# Autodesk Inventor assembly: 2020-2040_right
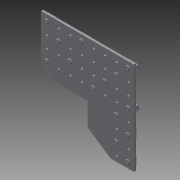
[picture p0: Inventor's stored thumbnail of the model, 180x180]
Saved by Autodesk Inventor 2014 (Build 180170000, 170)
## iProperties
Created: 2014-10-05
Part Number: 2020-2040_right
Document SubType Name: Assembly
Designer: Matthew
Author: Matthew
## Documents named in this file (3)
- C:\Users\Matthew\Documents\GitHub\CNC Mill\8020\2020-2040_right.iam
- C:\Users\Matthew\Documents\GitHub\CNC Mill\8020\2020-2040_mounting_plate.ipt
- C:\Users\Matthew\Documents\GitHub\CNC Mill\8020\0.5in_tnut.iam
## Components (15 placed, 2 different names)
1. 2020-2040_mounting_plate:1 — Insert:1, Insert:16, Insert:17, Insert:18, Insert:19, Insert:20, Insert:21, Insert:22, Insert:23, Insert:24, Insert:25, Insert:26, Insert:27, Insert:28
2. 0.5in_tnut:8 [sub-assembly] — Insert:17, Flush:2
3. 0.5in_tnut:13 [sub-assembly] — Insert:1
4. 0.5in_tnut:16 [sub-assembly] — Insert:16
5. 0.5in_tnut:18 [sub-assembly] — Insert:20, Flush:3
6. 0.5in_tnut:19 [sub-assembly] — Insert:18, Flush:3
7. 0.5in_tnut:20 [sub-assembly] — Insert:19, Flush:2
8. 0.5in_tnut:21 [sub-assembly] — Insert:21
9. 0.5in_tnut:22 [sub-assembly] — Insert:23
10. 0.5in_tnut:23 [sub-assembly] — Insert:22
11. 0.5in_tnut:24 [sub-assembly] — Insert:27
12. 0.5in_tnut:25 [sub-assembly] — Insert:26
13. 0.5in_tnut:26 [sub-assembly] — Insert:25
14. 0.5in_tnut:27 [sub-assembly] — Insert:24
15. 0.5in_tnut:28 [sub-assembly] — Insert:28
## Relationships (16: Insert 14, Flush 2)
- Insert:1: 2020-2040_mounting_plate:1 ↔ 0.5in_tnut:13
- Insert:16: 2020-2040_mounting_plate:1 ↔ 0.5in_tnut:16
- Insert:17: 2020-2040_mounting_plate:1 ↔ 0.5in_tnut:8
- Insert:18: 2020-2040_mounting_plate:1 ↔ 0.5in_tnut:19
- Insert:19: 2020-2040_mounting_plate:1 ↔ 0.5in_tnut:20
- Insert:20: 2020-2040_mounting_plate:1 ↔ 0.5in_tnut:18
- Flush:2: 0.5in_tnut:8 ↔ 0.5in_tnut:20
- Flush:3: 0.5in_tnut:18 ↔ 0.5in_tnut:19
- Insert:21: 2020-2040_mounting_plate:1 ↔ 0.5in_tnut:21
- Insert:22: 2020-2040_mounting_plate:1 ↔ 0.5in_tnut:23
- Insert:23: 2020-2040_mounting_plate:1 ↔ 0.5in_tnut:22
- Insert:24: 2020-2040_mounting_plate:1 ↔ 0.5in_tnut:27
- Insert:25: 2020-2040_mounting_plate:1 ↔ 0.5in_tnut:26
- Insert:26: 2020-2040_mounting_plate:1 ↔ 0.5in_tnut:25
- Insert:27: 2020-2040_mounting_plate:1 ↔ 0.5in_tnut:24
- Insert:28: 2020-2040_mounting_plate:1 ↔ 0.5in_tnut:28
